# Autodesk Inventor assembly: Track Idler Assembly
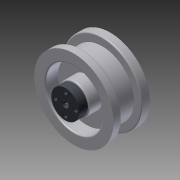
[picture p0: Inventor's stored thumbnail of the model, 180x180]
Saved by Autodesk Inventor 2015 (Build 190159000, 159)
## iProperties
Created: 2015-09-26
Part Number: Track Idler Assembly
Document SubType Name: Assembly
Designer: Jing-Chen
Author: Jing-Chen
## Documents named in this file (5)
- C:\Users\Jing-Chen\Desktop\Bionic Hybrids 2016\Bionic-Hybrids\CAD\Drivetrain\Sub-Assemblies\Track Idler Assembly.iam
- C:\Users\Jing-Chen\Desktop\Bionic Hybrids 2016\Bionic-Hybrids\Stock\Track Idler - 73646.ipt
- C:\Users\Jing-Chen\Desktop\Bionic Hybrids 2016\Bionic-Hybrids\Stock\Shaft Collar-Setscrew, Axle, Mountable - 739172.iam
- C:\Users\Jing-Chen\Desktop\Bionic Hybrids 2016\Bionic-Hybrids\Stock\Bearing-Thrust - 739091.ipt
- C:\Users\Jing-Chen\Desktop\Bionic Hybrids 2016\Bionic-Hybrids\Stock\Screw 1.25in - 739194.ipt
## Components (7 placed, 4 different names)
1. Track Idler - 73646:1 — Mate:1, Mate:2, Mate:3, Mate:4, Mate:5, Mate:6, Mate:7, Mate:8, Mate:9, Mate:10, Mate:11, Mate:12, Mate:13
2. Shaft Collar-Setscrew, Axle, Mountable - 739172:1 [sub-assembly] — Mate:1, Mate:2, Mate:3
3. Bearing-Thrust - 739091:1 — Mate:4, Mate:5
4. Screw 1.25in - 739194:1 — Mate:7, Mate:11
5. Screw 1.25in - 739194:2 — Mate:9, Mate:13
6. Screw 1.25in - 739194:3 — Mate:8, Mate:12
7. Screw 1.25in - 739194:4 — Mate:6, Mate:10
## Relationships (13: Mate 13)
- Mate:1: Track Idler - 73646:1 ↔ Shaft Collar-Setscrew, Axle, Mountable - 739172:1
- Mate:2: Track Idler - 73646:1 ↔ Shaft Collar-Setscrew, Axle, Mountable - 739172:1
- Mate:3: Track Idler - 73646:1 ↔ Shaft Collar-Setscrew, Axle, Mountable - 739172:1
- Mate:4: Track Idler - 73646:1 ↔ Bearing-Thrust - 739091:1
- Mate:5: Track Idler - 73646:1 ↔ Bearing-Thrust - 739091:1
- Mate:6: Track Idler - 73646:1 ↔ Screw 1.25in - 739194:4
- Mate:7: Track Idler - 73646:1 ↔ Screw 1.25in - 739194:1
- Mate:8: Track Idler - 73646:1 ↔ Screw 1.25in - 739194:3
- Mate:9: Track Idler - 73646:1 ↔ Screw 1.25in - 739194:2
- Mate:10: Track Idler - 73646:1 ↔ Screw 1.25in - 739194:4
- Mate:11: Track Idler - 73646:1 ↔ Screw 1.25in - 739194:1
- Mate:12: Track Idler - 73646:1 ↔ Screw 1.25in - 739194:3
- Mate:13: Track Idler - 73646:1 ↔ Screw 1.25in - 739194:2
